# Autodesk Inventor assembly: tau2
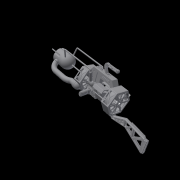
[picture p0: Inventor's stored thumbnail of the model, 180x180]
Saved by Autodesk Inventor 2020.4 (Build 244396010, 396A)
## iProperties
Created: 2022-09-08
Part Number: tau2
Document SubType Name: Assembly
Designer: Val
Author: Val
## Documents named in this file (30)
- C:\Users\Val\Desktop\tau\Tau.iam
- C:\Users\Val\Desktop\tau\external\TopHandle.ipt
- C:\Users\Val\Desktop\tau\Body.ipt
- C:\Users\Val\Desktop\tau\external\FlowMeter.ipt
- C:\Users\Val\Desktop\tau\external\SideHandle.ipt
- C:\Users\Val\Desktop\tau\external\SideHandleBase.ipt
- C:\Users\Val\Desktop\tau\HexCoil.ipt
- C:\Users\Val\Desktop\tau\CoilCover.ipt
- C:\Users\Val\Desktop\tau\Stock.ipt
- C:\Users\Val\Desktop\tau\Stock_MIR.ipt
- C:\Users\Val\Desktop\tau\HoseConnector.ipt
- C:\Users\Val\Desktop\tau\BatteryCover.ipt
- C:\Users\Val\Desktop\tau\BatteryCoverLid.ipt
- C:\Users\Val\Desktop\tau\MuzzleTube.ipt
- C:\Users\Val\Desktop\tau\MuzzleEndBall.ipt
- C:\Users\Val\Desktop\tau\MuzzleEndTube.ipt
- C:\Users\Val\Desktop\tau\ToroidalCore.ipt
- C:\Users\Val\Desktop\tau\MuzzleWireProtector.ipt
- C:\Users\Val\Desktop\tau\TopPipe.ipt
- C:\Users\Val\Desktop\tau\external\CO2Cartridge16g.ipt
- C:\Users\Val\Desktop\tau\external\Picatinny6.ipt
- C:\Users\Val\Desktop\tau\BatteryHeatsink.ipt
- C:\Users\Val\Desktop\tau\StockMountPlate.ipt
- C:\Users\Val\Desktop\tau\BodyMirror.ipt
- C:\Users\Val\Desktop\tau\TopPipeStraight.ipt
- C:\Users\Val\Desktop\tau\BatteryPlate.ipt
- C:\Users\Val\Desktop\tau\StockBack.ipt
- C:\Users\Val\Desktop\tau\external\CO2FeedPipe.ipt
- C:\Users\Val\Desktop\tau\external\Picatinny10.ipt
- C:\Users\Val\Desktop\tau\external\Picatinny14.ipt
## Components (43 placed, 29 different names)
1. TopHandle:1
2. Body:1 — Mate:1, Mate:3, Mate:4, Mate:6, Mate:15, Mate:26, Mate:30, Flush:35, Mate:37, Mate:38, Mate:56, Mate:79, Mate:80, Mate:81, Mate:98, Mate:100, Angle:7, Flush:48, Mate:103
3. FlowMeter:1 — Mate:3, Mate:4, Mate:6
4. SideHandle:1 — Mate:52, Mate:53
5. HexCoil:1 — Mate:13, Mate:15, Flush:6, Flush:7, Mate:27, Flush:10, Flush:11, Mate:31, Flush:12, Flush:13, Flush:37, Angle:1, Angle:2
6. HexCoil:2 — Flush:6, Flush:7, Mate:22, Flush:8, Mate:24, Flush:9, Mate:25, Flush:35, Mate:72, Mate:73, Mate:74
7. CoilCover:1 — Mate:22, Flush:8, Mate:25, Mate:45
8. CoilCover:2 — Mate:24, Flush:9, Mate:26
9. CoilCover:3 — Mate:31, Flush:12, Flush:13, Flush:36, Mate:33
10. CoilCover:4 — Mate:27, Flush:10, Flush:11, Mate:30
11. Stock:1 — Flush:34, Mate:75, Mate:76, Mate:95, Mate:96, Mate:105
12. Stock_MIR:1 — Mate:77, Mate:78, Mate:106
13. HoseConnector:1 — Flush:36, Mate:33, Flush:37
14. BatteryCover:1 — Flush:38, Flush:39, Flush:44, Flush:45, Mate:66, Mate:67, Mate:68, Mate:85, Mate:86, Mate:87
15. BatteryCover:2 — Flush:38, Mate:35, Flush:40, Flush:41, Mate:64, Mate:65, Angle:6, Mate:88, Mate:89, Mate:90
16. BatteryCover:3 — Flush:39, Mate:36, Flush:42, Flush:43, Mate:39, Flush:46, Flush:47, Mate:69, Mate:70, Mate:71, Mate:91, Mate:92, Mate:93
17. BatteryCoverLid:1 — Mate:35, Flush:40, Flush:41, Mate:36, Flush:42, Flush:43, Flush:44, Flush:45, Mate:37, Mate:38
18. BatteryCoverLid:2 — Mate:39, Flush:46, Flush:47
19. MuzzleTube:1 — Mate:42, Mate:46
20. MuzzleEndBall:1 — Mate:43, Mate:44, Mate:48
21. MuzzleEndTube:1 — Mate:42, Mate:43, Angle:1, Angle:2, Mate:44, Mate:48
22. ToroidalCore:1 — Mate:46
23. ToroidalCore:2 — Mate:45
24. MuzzleWireProtector:1
25. TopPipe:1
26. CO2Cartridge16g:1 — Mate:94
27. Picatinny6:2 — Mate:56, Mate:98, Mate:99
28. SideHandleBase:1 — Mate:52, Mate:53, Mate:107, Mate:108
29. BatteryHeatsink:1 — Mate:64, Mate:65, Angle:6
30. BatteryHeatsink:2 — Mate:66, Mate:67, Mate:68
31. BatteryHeatsink:3 — Mate:69, Mate:70, Mate:71
32. StockMountPlate:1 — Mate:72, Mate:73, Mate:74, Mate:75, Mate:76, Mate:77, Mate:78
33. BodyMirror:1 — Mate:79, Mate:80, Mate:81, Mate:99, Mate:101, Angle:8, Flush:49, Mate:102, Flush:51
34. TopPipeStraight:1 — Mate:94
35. BatteryPlate:1 — Mate:85, Mate:86, Mate:87
36. BatteryPlate:2 — Mate:88, Mate:89, Mate:90
37. BatteryPlate:3 — Mate:91, Mate:92, Mate:93
38. StockBack:1 — Mate:95, Mate:96
39. CO2FeedPipe:1
40. Picatinny10:1 — Mate:100, Angle:7, Flush:48, Flush:50, Mate:107, Mate:108
41. Picatinny10:2 — Mate:101, Angle:8, Flush:49, Flush:50
42. Picatinny14:1 — Mate:104, Mate:105, Mate:106
43. Picatinny10:3 — Mate:102, Mate:103, Flush:51
## Relationships (101: Mate 69, Flush 26, Angle 5, Symmetry 1)
- Symmetry:1
- Mate:1: Body:1
- Mate:3: Body:1 ↔ FlowMeter:1
- Mate:4: Body:1 ↔ FlowMeter:1
- Mate:6: Body:1 ↔ FlowMeter:1
- Mate:13: HexCoil:1
- Mate:15: Body:1 ↔ HexCoil:1
- Flush:6: HexCoil:1 ↔ HexCoil:2
- Flush:7: HexCoil:1 ↔ HexCoil:2
- Mate:22: HexCoil:2 ↔ CoilCover:1
- Flush:8: HexCoil:2 ↔ CoilCover:1
- Mate:24: HexCoil:2 ↔ CoilCover:2
- Flush:9: HexCoil:2 ↔ CoilCover:2
- Mate:25: HexCoil:2 ↔ CoilCover:1
- Mate:26: Body:1 ↔ CoilCover:2
- Mate:27: HexCoil:1 ↔ CoilCover:4
- Flush:10: HexCoil:1 ↔ CoilCover:4
- Flush:11: HexCoil:1 ↔ CoilCover:4
- Mate:30: Body:1 ↔ CoilCover:4
- Mate:31: HexCoil:1 ↔ CoilCover:3
- Flush:12: HexCoil:1 ↔ CoilCover:3
- Flush:13: HexCoil:1 ↔ CoilCover:3
- Flush:34: Stock:1
- Flush:35: Body:1 ↔ HexCoil:2
- Flush:36: CoilCover:3 ↔ HoseConnector:1
- Mate:33: CoilCover:3 ↔ HoseConnector:1
- Flush:37: HexCoil:1 ↔ HoseConnector:1
- Flush:38: BatteryCover:1 ↔ BatteryCover:2
- Flush:39: BatteryCover:1 ↔ BatteryCover:3
- Mate:35: BatteryCover:2 ↔ BatteryCoverLid:1
- Flush:40: BatteryCover:2 ↔ BatteryCoverLid:1
- Flush:41: BatteryCover:2 ↔ BatteryCoverLid:1
- Mate:36: BatteryCover:3 ↔ BatteryCoverLid:1
- Flush:42: BatteryCover:3 ↔ BatteryCoverLid:1
- Flush:43: BatteryCover:3 ↔ BatteryCoverLid:1
- Flush:44: BatteryCover:1 ↔ BatteryCoverLid:1
- Flush:45: BatteryCover:1 ↔ BatteryCoverLid:1
- Mate:37: Body:1 ↔ BatteryCoverLid:1
- Mate:38: Body:1 ↔ BatteryCoverLid:1
- Mate:39: BatteryCover:3 ↔ BatteryCoverLid:2
- Flush:46: BatteryCover:3 ↔ BatteryCoverLid:2
- Flush:47: BatteryCover:3 ↔ BatteryCoverLid:2
- Mate:42: MuzzleTube:1 ↔ MuzzleEndTube:1
- Mate:43: MuzzleEndBall:1 ↔ MuzzleEndTube:1
- Angle:1 (0 deg): HexCoil:1 ↔ MuzzleEndTube:1
- Angle:2 (0 deg): HexCoil:1 ↔ MuzzleEndTube:1
- Mate:44: MuzzleEndBall:1 ↔ MuzzleEndTube:1
- Mate:45: CoilCover:1 ↔ ToroidalCore:2
- Mate:46: MuzzleTube:1 ↔ ToroidalCore:1
- Mate:48: MuzzleEndBall:1 ↔ MuzzleEndTube:1
- Mate:52: SideHandle:1 ↔ SideHandleBase:1
- Mate:53: SideHandle:1 ↔ SideHandleBase:1
- Mate:56: Body:1 ↔ Picatinny6:2
- Mate:64: BatteryCover:2 ↔ BatteryHeatsink:1
- Mate:65: BatteryCover:2 ↔ BatteryHeatsink:1
- Angle:6 (0 deg): BatteryCover:2 ↔ BatteryHeatsink:1
- Mate:66: BatteryCover:1 ↔ BatteryHeatsink:2
- Mate:67: BatteryCover:1 ↔ BatteryHeatsink:2
- Mate:68: BatteryCover:1 ↔ BatteryHeatsink:2
- Mate:69: BatteryCover:3 ↔ BatteryHeatsink:3
- Mate:70: BatteryCover:3 ↔ BatteryHeatsink:3
- Mate:71: BatteryCover:3 ↔ BatteryHeatsink:3
- Mate:72: HexCoil:2 ↔ StockMountPlate:1
- Mate:73: HexCoil:2 ↔ StockMountPlate:1
- Mate:74: HexCoil:2 ↔ StockMountPlate:1
- Mate:75: Stock:1 ↔ StockMountPlate:1
- Mate:76: Stock:1 ↔ StockMountPlate:1
- Mate:77: Stock_MIR:1 ↔ StockMountPlate:1
- Mate:78: Stock_MIR:1 ↔ StockMountPlate:1
- Mate:79: Body:1 ↔ BodyMirror:1
- Mate:80: Body:1 ↔ BodyMirror:1
- Mate:81: Body:1 ↔ BodyMirror:1
- Mate:85: BatteryCover:1 ↔ BatteryPlate:1
- Mate:86: BatteryCover:1 ↔ BatteryPlate:1
- Mate:87: BatteryCover:1 ↔ BatteryPlate:1
- Mate:88: BatteryCover:2 ↔ BatteryPlate:2
- Mate:89: BatteryCover:2 ↔ BatteryPlate:2
- Mate:90: BatteryCover:2 ↔ BatteryPlate:2
- Mate:91: BatteryCover:3 ↔ BatteryPlate:3
- Mate:92: BatteryCover:3 ↔ BatteryPlate:3
- Mate:93: BatteryCover:3 ↔ BatteryPlate:3
- Mate:94: CO2Cartridge16g:1 ↔ TopPipeStraight:1
- Mate:95: Stock:1 ↔ StockBack:1
- Mate:96: Stock:1 ↔ StockBack:1
- Mate:98: Body:1 ↔ Picatinny6:2
- Mate:99 (8.4667 mm): Picatinny6:2 ↔ BodyMirror:1
- Mate:100: Body:1 ↔ Picatinny10:1
- Angle:7 (0 deg): Body:1 ↔ Picatinny10:1
- Flush:48 (-5 mm): Body:1 ↔ Picatinny10:1
- Mate:101: BodyMirror:1 ↔ Picatinny10:2
- Angle:8 (0 deg): BodyMirror:1 ↔ Picatinny10:2
- Flush:49 (5 mm): BodyMirror:1 ↔ Picatinny10:2
- Flush:50: Picatinny10:1 ↔ Picatinny10:2
- Mate:102: BodyMirror:1 ↔ Picatinny10:3
- Mate:103: Body:1 ↔ Picatinny10:3
- Flush:51 (-5 mm): BodyMirror:1 ↔ Picatinny10:3
- Mate:104: Picatinny14:1
- Mate:105: Stock:1 ↔ Picatinny14:1
- Mate:106 (6 mm): Stock_MIR:1 ↔ Picatinny14:1
- Mate:107: SideHandleBase:1 ↔ Picatinny10:1
- Mate:108: SideHandleBase:1 ↔ Picatinny10:1
